# Autodesk Inventor assembly: assembly
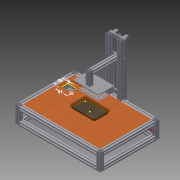
[picture p0: Inventor's stored thumbnail of the model, 180x180]
Saved by Autodesk Inventor 2015 SP1 (Build 190203100, 203)
## iProperties
Created: 2015-04-22
Part Number: assembly
Document SubType Name: Assembly
Designer: ubik
Author: ubik
## Documents named in this file (26)
- C:\Users\ubik\Dropbox\DueTech\cable test\assembly.iam
- C:\Users\ubik\Dropbox\DueTech\cable test\20.1068-30X30-3.ipt
- C:\Users\ubik\Dropbox\DueTech\cable test\20.1068-30X30-3\20.1068-30X30-400.ipt
- C:\Users\ubik\Dropbox\DueTech\cable test\20.1068-30X30-3\20.1068-30X30-600.ipt
- C:\Users\ubik\Dropbox\DueTech\cable test\top plate.ipt
- C:\Users\ubik\Dropbox\proiecte\inventor\inventor library\sk12.ipt
- C:\Users\ubik\Dropbox\DueTech\cable test\linear shaft.ipt
- C:\Users\ubik\Dropbox\DueTech\cable test\motor plate support.ipt
- C:\Users\ubik\Dropbox\proiecte\inventor\inventor library\PM Wantai 811  Nema 17.ipt
- C:\Users\ubik\Dropbox\proiecte\inventor\inventor library\T2.5-12-3.0 Pulley.ipt
- C:\Users\ubik\Dropbox\DueTech\cable test\mobile plate.ipt
- C:\Users\ubik\Dropbox\DueTech\cable test\linear shaft\Shaft 12 450.ipt
- C:\Users\ubik\Dropbox\DueTech\cable test\alu top plate.ipt
- C:\Users\ubik\Dropbox\DueTech\cable test\20.1068-30X30-3\20.1068-30X30-200.ipt
- C:\Users\ubik\Documents\Inventor\Content Center Files\R2015\en-US\ANSI B18.3.1M(1)\ANSI B18.3.1M - M8x1.25 x 20(2).ipt
- C:\Users\ubik\Dropbox\DueTech\cable test\T2.5 belt\T2.5 belt-10.ipt
- C:\Users\ubik\Dropbox\DueTech\cable test\T2.5 belt.ipt
- C:\Users\ubik\Dropbox\DueTech\cable test\belt fixture.iam
- C:\Users\ubik\Dropbox\DueTech\cable test\cuva.ipt
- C:\Users\ubik\Dropbox\DueTech\cable test\20.1068-30X30-3\20.1068-30X30-130.ipt
- C:\Users\ubik\Dropbox\DueTech\cable test\20.1068-30X30-3\20.1068-30X30-100.ipt
- C:\Users\ubik\Dropbox\DueTech\cable test\bearing 608.ipt
- C:\Users\ubik\Dropbox\DueTech\cable test\placa spate.ipt
- C:\Users\ubik\Dropbox\DueTech\cable test\capac cu gaura.ipt
- C:\Users\ubik\Dropbox\DueTech\cable test\capac 2.ipt
- C:\Users\ubik\Dropbox\DueTech\cable test\sita.ipt
## Components (37 placed, 22 different names)
1. 20.1068-30X30-130:1 — Flush:51, Mate:75, Flush:93, Flush:94, Flush:95, Mate:77, Mate:81, Flush:102, Flush:103, Flush:104, Mate:82
2. 20.1068-30X30-130:2 — Flush:53, Flush:54, Mate:76, Flush:96, Mate:80, Flush:99, Flush:100, Flush:101
3. 20.1068-30X30-130:3 — Flush:32, Mate:78, Mate:79, Flush:97, Flush:105
4. 20.1068-30X30-130:4 — Flush:40, Mate:73, Mate:74, Flush:92, Flush:98, Flush:108
5. 20.1068-30X30-400:5 — Flush:101, Mate:81, Flush:102
6. 20.1068-30X30-400:6 — Flush:49, Flush:51, Flush:54, Mate:76, Flush:95, Flush:96, Mate:77, Flush:110
7. 20.1068-30X30-600:7 — Flush:44, Mate:80, Flush:99, Flush:100
8. 20.1068-30X30-600:8 — Flush:46, Flush:74, Mate:45, Flush:103, Flush:104, Mate:82
9. 20.1068-30X30-600:9 — Flush:37, Mate:29, Flush:55, Mate:74, Flush:92, Mate:75, Flush:93, Flush:94, Flush:98, Mate:84
10. 20.1068-30X30-600:10 — Mate:16, Flush:49, Flush:53, Mate:78, Flush:97, Mate:90
11. 20.1068-30X30-400:11 — Flush:44, Flush:46, Flush:105
12. 20.1068-30X30-400:12 — Mate:16, Flush:32, Flush:37, Flush:40, Mate:73, Mate:79, Mate:83, Flush:106, Flush:109
13. top plate:1 — Mate:83, Mate:84, Flush:106
14. 20.1068-30X30-400:13 — Flush:30, Flush:56, Flush:57, Mate:30
15. 20.1068-30X30-400:14 — Flush:30, Mate:29, Flush:55, Flush:56, Flush:57, Mate:30, Flush:75, Flush:87, Mate:62, Flush:88, Flush:89, Angle:3, Flush:108
16. sk12:1 — Mate:32, Flush:61, Flush:67, Flush:77, Flush:85, Flush:86
17. sk12:2 — Mate:33, Flush:60, Flush:66, Flush:76, Mate:48, Flush:85, Flush:86
18. sk12:3 — Mate:34, Flush:60, Mate:38, Flush:87
19. sk12:4 — Mate:35, Flush:61, Flush:68
20. Shaft 12 450:1 — Mate:32, Mate:35, Flush:67, Flush:68
21. Shaft 12 450:2 — Mate:33, Mate:34, Flush:66, Mate:38
22. PM Wantai 811  Nema 17:1 — Mate:43, Mate:44, Mate:46, Mate:47, Mate:55
23. T2.5-12-3.0 Pulley:1 — Mate:43, Mate:44
24. motor plate support:1 — Flush:74, Mate:45, Flush:75, Mate:46, Mate:47, Flush:76, Flush:77, Mate:48, Mate:55
25. mobile plate:1 — Mate:66, Mate:85, Flush:107
26. alu top plate:1 — Mate:62, Flush:88, Flush:89, Mate:86
27. 20.1068-30X30-200:15 — Flush:90, Flush:91, Mate:65, Mate:66, Angle:3
28. 20.1068-30X30-100:16 — Flush:90, Flush:91, Mate:65, Mate:91, Mate:92, Angle:5
29. Broached Socket Head Cap Screw - Metric M8x1.25 x 20:1
30. T2.5 belt-10:2
31. cuva:1 — Flush:109
32. belt fixture:1 [sub-assembly] — Mate:85, Flush:107
33. bearing 608:1 — Mate:86
34. placa spate:1
35. capac cu gaura:1 — Mate:90, Flush:110
36. capac 2:1 — Mate:91, Mate:92, Angle:5, Flush:111
37. sita:1 — Flush:111
## Relationships (86: Flush 49, Mate 35, Angle 2)
- Flush:30: 20.1068-30X30-400:13 ↔ 20.1068-30X30-400:14
- Mate:16: 20.1068-30X30-600:10 ↔ 20.1068-30X30-400:12
- Flush:32: 20.1068-30X30-130:3 ↔ 20.1068-30X30-400:12
- Flush:37: 20.1068-30X30-600:9 ↔ 20.1068-30X30-400:12
- Flush:40: 20.1068-30X30-130:4 ↔ 20.1068-30X30-400:12
- Flush:44: 20.1068-30X30-600:7 ↔ 20.1068-30X30-400:11
- Flush:46: 20.1068-30X30-600:8 ↔ 20.1068-30X30-400:11
- Flush:49: 20.1068-30X30-400:6 ↔ 20.1068-30X30-600:10
- Flush:51: 20.1068-30X30-130:1 ↔ 20.1068-30X30-400:6
- Flush:53: 20.1068-30X30-130:2 ↔ 20.1068-30X30-600:10
- Flush:54: 20.1068-30X30-130:2 ↔ 20.1068-30X30-400:6
- Mate:29: 20.1068-30X30-600:9 ↔ 20.1068-30X30-400:14
- Flush:55: 20.1068-30X30-600:9 ↔ 20.1068-30X30-400:14
- Flush:56: 20.1068-30X30-400:13 ↔ 20.1068-30X30-400:14
- Flush:57: 20.1068-30X30-400:13 ↔ 20.1068-30X30-400:14
- Mate:30 (60 mm): 20.1068-30X30-400:13 ↔ 20.1068-30X30-400:14
- Mate:32: sk12:1 ↔ Shaft 12 450:1
- Mate:33: sk12:2 ↔ Shaft 12 450:2
- Mate:34: sk12:3 ↔ Shaft 12 450:2
- Mate:35: sk12:4 ↔ Shaft 12 450:1
- Flush:60: sk12:2 ↔ sk12:3
- Flush:61: sk12:1 ↔ sk12:4
- Flush:66: sk12:2 ↔ Shaft 12 450:2
- Flush:67: sk12:1 ↔ Shaft 12 450:1
- Mate:38: sk12:3 ↔ Shaft 12 450:2
- Flush:68: sk12:4 ↔ Shaft 12 450:1
- Mate:43: PM Wantai 811  Nema 17:1 ↔ T2.5-12-3.0 Pulley:1
- Mate:44 (5 mm): PM Wantai 811  Nema 17:1 ↔ T2.5-12-3.0 Pulley:1
- Flush:74: 20.1068-30X30-600:8 ↔ motor plate support:1
- Mate:45: 20.1068-30X30-600:8 ↔ motor plate support:1
- Flush:75: 20.1068-30X30-400:14 ↔ motor plate support:1
- Mate:46: PM Wantai 811  Nema 17:1 ↔ motor plate support:1
- Mate:47: PM Wantai 811  Nema 17:1 ↔ motor plate support:1
- Flush:76: sk12:2 ↔ motor plate support:1
- Flush:77: sk12:1 ↔ motor plate support:1
- Mate:48: sk12:2 ↔ motor plate support:1
- Mate:55: PM Wantai 811  Nema 17:1 ↔ motor plate support:1
- Flush:85: sk12:1 ↔ sk12:2
- Flush:86: sk12:1 ↔ sk12:2
- Flush:87: 20.1068-30X30-400:14 ↔ sk12:3
- Mate:62: 20.1068-30X30-400:14 ↔ alu top plate:1
- Flush:88: 20.1068-30X30-400:14 ↔ alu top plate:1
- Flush:89: 20.1068-30X30-400:14 ↔ alu top plate:1
- Flush:90: 20.1068-30X30-200:15 ↔ 20.1068-30X30-100:16
- Flush:91: 20.1068-30X30-200:15 ↔ 20.1068-30X30-100:16
- Mate:65: 20.1068-30X30-200:15 ↔ 20.1068-30X30-100:16
- Mate:66: mobile plate:1 ↔ 20.1068-30X30-200:15
- Angle:3 (0 deg): 20.1068-30X30-400:14 ↔ 20.1068-30X30-200:15
- Mate:73: 20.1068-30X30-130:4 ↔ 20.1068-30X30-400:12
- Mate:74: 20.1068-30X30-130:4 ↔ 20.1068-30X30-600:9
- Flush:92: 20.1068-30X30-130:4 ↔ 20.1068-30X30-600:9
- Mate:75: 20.1068-30X30-130:1 ↔ 20.1068-30X30-600:9
- Flush:93: 20.1068-30X30-130:1 ↔ 20.1068-30X30-600:9
- Flush:94: 20.1068-30X30-130:1 ↔ 20.1068-30X30-600:9
- Mate:76: 20.1068-30X30-130:2 ↔ 20.1068-30X30-400:6
- Flush:95: 20.1068-30X30-130:1 ↔ 20.1068-30X30-400:6
- Flush:96: 20.1068-30X30-130:2 ↔ 20.1068-30X30-400:6
- Mate:77: 20.1068-30X30-130:1 ↔ 20.1068-30X30-400:6
- Mate:78: 20.1068-30X30-130:3 ↔ 20.1068-30X30-600:10
- Mate:79: 20.1068-30X30-130:3 ↔ 20.1068-30X30-400:12
- Flush:97: 20.1068-30X30-130:3 ↔ 20.1068-30X30-600:10
- Flush:98: 20.1068-30X30-130:4 ↔ 20.1068-30X30-600:9
- Mate:80: 20.1068-30X30-130:2 ↔ 20.1068-30X30-600:7
- Flush:99: 20.1068-30X30-130:2 ↔ 20.1068-30X30-600:7
- Flush:100: 20.1068-30X30-130:2 ↔ 20.1068-30X30-600:7
- Flush:101: 20.1068-30X30-130:2 ↔ 20.1068-30X30-400:5
- Mate:81: 20.1068-30X30-130:1 ↔ 20.1068-30X30-400:5
- Flush:102: 20.1068-30X30-130:1 ↔ 20.1068-30X30-400:5
- Flush:103: 20.1068-30X30-130:1 ↔ 20.1068-30X30-600:8
- Flush:104: 20.1068-30X30-130:1 ↔ 20.1068-30X30-600:8
- Mate:82: 20.1068-30X30-130:1 ↔ 20.1068-30X30-600:8
- Flush:105: 20.1068-30X30-130:3 ↔ 20.1068-30X30-400:11
- Mate:83: 20.1068-30X30-400:12 ↔ top plate:1
- Mate:84: 20.1068-30X30-600:9 ↔ top plate:1
- Flush:106: 20.1068-30X30-400:12 ↔ top plate:1
- Mate:85: mobile plate:1 ↔ belt fixture:1
- Mate:86: alu top plate:1 ↔ bearing 608:1
- Flush:107: mobile plate:1 ↔ belt fixture:1
- Flush:108 (270 mm): 20.1068-30X30-130:4 ↔ 20.1068-30X30-400:14
- Flush:109 (231.25 mm): 20.1068-30X30-400:12 ↔ cuva:1
- Mate:90: 20.1068-30X30-600:10 ↔ capac cu gaura:1
- Flush:110: 20.1068-30X30-400:6 ↔ capac cu gaura:1
- Mate:91: 20.1068-30X30-100:16 ↔ capac 2:1
- Mate:92: 20.1068-30X30-100:16 ↔ capac 2:1
- Angle:5 (0 deg): 20.1068-30X30-100:16 ↔ capac 2:1
- Flush:111 (60 mm): capac 2:1 ↔ sita:1
